# Autodesk Inventor assembly: Base_Assembly_V02
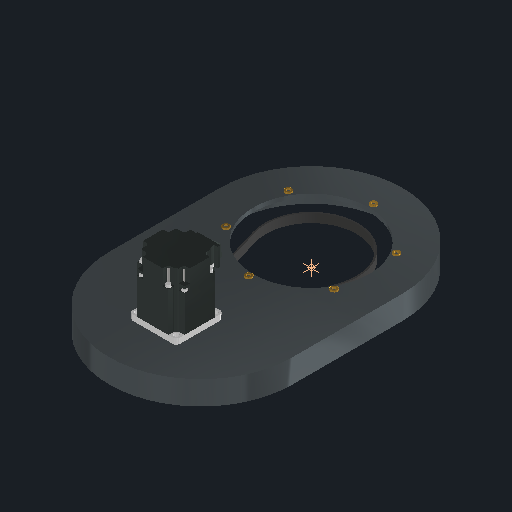
[picture p0: Inventor's stored thumbnail of the model, 512x512]
Saved by Autodesk Inventor 2026 (Build 300175000, 175)
## iProperties
Created: 2025-12-01
Part Number: Base_Assembly_V02
Document SubType Name: Assembly
Designer: DanielFGarzon
Mass: 1482.32 g
Surface Area: 2260.79 cm^2
Volume: 923.556 cm^3
Density: 1.60501 g/cm^3
Author: DanielFGarzon
## Documents named in this file (6)
- D:\POLIMI\3RD SEMESTER\Industrial Robotics\Project\Mine\Base_Assembly_V02.iam
- D:\POLIMI\3RD SEMESTER\Industrial Robotics\Project\Mine\BASE.ipt
- D:\POLIMI\3RD SEMESTER\Industrial Robotics\Project\Mine\Motor_02.ipt
- D:\POLIMI\3RD SEMESTER\Industrial Robotics\Project\Mine\3M120T_03.ipt
- D:\POLIMI\3RD SEMESTER\Industrial Robotics\Project\Mine\Belt_03.ipt
- D:\POLIMI\3RD SEMESTER\Industrial Robotics\Project\Mine\Spacer_05.ipt
## Components (10 placed, 5 different names)
1. BASE:1 — Mate:1, Mate:2, Mate:3, Mate:4, Mate:8, Mate:9, Mate:10, Mate:11, Mate:12, Mate:13, Mate:14, Mate:15, Mate:16, Mate:17, Mate:18, Mate:19, Mate:20, Flush:1
2. Motor_02:1 — Mate:3, Mate:4, Mate:5, Mate:21
3. 3M120T_03:1 — Mate:5, Mate:6, Flush:1
4. Belt_03:1 — Mate:6, Mate:8, Mate:21
5. Spacer_05:1 — Mate:9, Mate:20
6. Spacer_05:2 — Mate:13, Mate:15
7. Spacer_05:3 — Mate:10, Mate:19
8. Spacer_05:4 — Mate:12, Mate:16
9. Spacer_05:5 — Mate:14, Mate:18
10. Spacer_05:6 — Mate:11, Mate:17
## Relationships (21: Mate 20, Flush 1)
- Mate:1: BASE:1
- Mate:2: BASE:1
- Mate:3: BASE:1 ↔ Motor_02:1
- Mate:4: BASE:1 ↔ Motor_02:1
- Mate:5: Motor_02:1 ↔ 3M120T_03:1
- Mate:6: 3M120T_03:1 ↔ Belt_03:1
- Mate:8: BASE:1 ↔ Belt_03:1
- Mate:9: BASE:1 ↔ Spacer_05:1
- Mate:10: BASE:1 ↔ Spacer_05:3
- Mate:11: BASE:1 ↔ Spacer_05:6
- Mate:12: BASE:1 ↔ Spacer_05:4
- Mate:13: BASE:1 ↔ Spacer_05:2
- Mate:14: BASE:1 ↔ Spacer_05:5
- Mate:15: BASE:1 ↔ Spacer_05:2
- Mate:16: BASE:1 ↔ Spacer_05:4
- Mate:17: BASE:1 ↔ Spacer_05:6
- Mate:18: BASE:1 ↔ Spacer_05:5
- Mate:19: BASE:1 ↔ Spacer_05:3
- Mate:20: BASE:1 ↔ Spacer_05:1
- Mate:21: Motor_02:1 ↔ Belt_03:1
- Flush:1 (-18 mm): BASE:1 ↔ 3M120T_03:1
